# Autodesk Inventor assembly: Feather_0_assembly
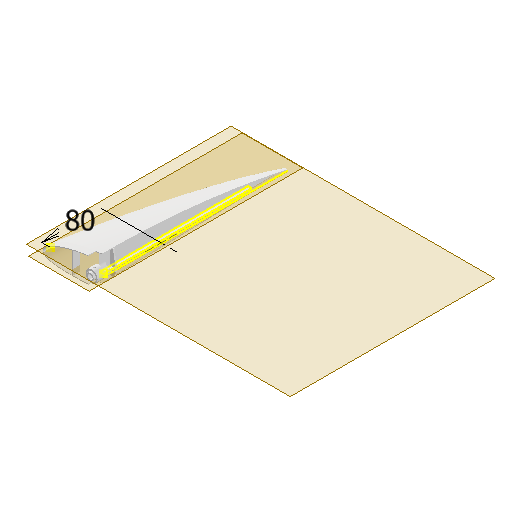
[picture p0: Inventor's stored thumbnail of the model, 512x512]
Saved by Autodesk Inventor 2022 (Build 260153000, 153)
## iProperties
Created: 2022-09-03
Part Number: Feather_0_assembly
Document SubType Name: Assembly
Designer: dell
Author: dell
## Documents named in this file (4)
- D:\xxxx\Uni\Part IV\MECHENG_700\Part_IV_project_CAD\Bird_skeleton_prototypes\Wing_drone_V1\Bird_wing_V2\Feather_0\Feather_0_assembly.iam
- D:\xxxx\Uni\Part IV\MECHENG_700\Part_IV_project_CAD\Bird_skeleton_prototypes\Wing_drone_V1\Bird_wing_V2\Feather_0\Feather_0_aerofoil_frame.ipt
- D:\xxxx\Uni\Part IV\MECHENG_700\Part_IV_project_CAD\Bird_skeleton_prototypes\Wing_drone_V1\Bird_wing_V2\Feather_0\Feather_0_aerofoil_frame_support.ipt
- D:\xxxx\Uni\Part IV\MECHENG_700\Part_IV_project_CAD\Bird_skeleton_prototypes\Wing_drone_V1\Bird_wing_V2\Feather_0\Feather_0_aerofoil_frame_support_p2.ipt
## Components (3 placed, 3 different names)
1. Feather_0_aerofoil_frame:1 — Mate:1, Mate:2, Mate:3, Mate:4, Flush:1
2. Feather_0_aerofoil_frame_support:1 — Mate:1, Mate:2, Mate:3, Mate:5
3. Feather_0_aerofoil_frame_support_p2:1 — Mate:4, Mate:5
## Relationships (6: Mate 5, Flush 1)
- Mate:1: Feather_0_aerofoil_frame:1 ↔ Feather_0_aerofoil_frame_support:1
- Mate:2: Feather_0_aerofoil_frame:1 ↔ Feather_0_aerofoil_frame_support:1
- Mate:3: Feather_0_aerofoil_frame:1 ↔ Feather_0_aerofoil_frame_support:1
- Mate:4: Feather_0_aerofoil_frame:1 ↔ Feather_0_aerofoil_frame_support_p2:1
- Mate:5: Feather_0_aerofoil_frame_support:1 ↔ Feather_0_aerofoil_frame_support_p2:1
- Flush:1: Feather_0_aerofoil_frame:1
